# Autodesk Inventor assembly: FLUGGER POWER PNL ASSY
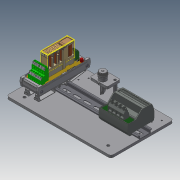
[picture p0: Inventor's stored thumbnail of the model, 180x180]
Saved by Autodesk Inventor 2020.3 (Build 243373000, 373)
## iProperties
RuleStatus: InUse
AfterDocSave0: file://Part Number Cleaner
Created: 2019-11-06
Vendor: HHMI: JRC - ID&F
Document SubType Name: Assembly
Designer: arnoldj
DESIGN DEPARTMENT: HHMI: JRC - ID&F
ALTERED ITEM PART NUMBER: N/A
ALTERED ITEM VENDOR: N/A
ALTERED ITEM DESCRIPTION: N/A
Author: arnoldj
Revision Number: 0
## Documents named in this file (9)
- C:\_WORKSPACE\DATA\PROJECTS\_PROJECTS BY LAB\CARD (LAB)\FLUGGER\FLUGGER POWER PNL ASSY.iam
- C:\_WORKSPACE\DATA\COMMON\Phoenix Contact\PHOENIX CONTACT 2315269 .ipt
- C:\_WORKSPACE\DATA\PROJECTS\_PROJECTS BY LAB\CARD (LAB)\FLUGGER\FLUGGER DIN RAIL MOUNT.ipt
- C:\_WORKSPACE\DATA\PROJECTS\_PROJECTS BY LAB\CARD (LAB)\FLUGGER\FLUGGER 8961K15 RAIL AI.ipt
- C:\_WORKSPACE\DATA\COMMON\Altech\Altech156.OA02.2433C.ipt
- C:\_WORKSPACE\DATA\PROJECTS\_PROJECTS BY LAB\CARD (LAB)\FLUGGER\FLUGGER FUSE MOUNT.ipt
- C:\_WORKSPACE\DATA\COMMON\McMaster\MCMASTER 7087K41 FUSEHOLDER .ipt
- C:\_WORKSPACE\DATA\COMMON\Littlefuse\Littlefuse 0218.315HXP.ipt
- C:\_WORKSPACE\DATA\COMMON\McMaster\MCMASTER 91115A146 STANDOFF 10-32x1_5L SS.ipt
## Components (9 placed, 8 different names)
1. FLUGGER DIN RAIL MOUNT:1 — Mate:1, Mate:2, Mate:3, Mate:4, Mate:7, Mate:10, Mate:11, Mate:12, Mate:16, Mate:18, Mate:19
2. PHOENIX CONTACT 2315269 :1 — Mate:5, Mate:6, Mate:7
3. FLUGGER 8961K15 RAIL AI:1 — Mate:1, Mate:2, Mate:3, Mate:4, Mate:5, Mate:6, Mate:8, Mate:9
4. Altech156.OA02.2433C:1 — Mate:8, Mate:9
5. FLUGGER FUSE MOUNT:1 — Mate:10, Mate:11, Mate:12, Mate:13, Mate:14, Mate:17
6. MCMASTER 7087K41 FUSEHOLDER :1 — Mate:13, Mate:14, Flush:1, Mate:15
7. Littlefuse 0218.315HXP:1 — Flush:1, Mate:15
8. MCMASTER 91115A146 STANDOFF 10-32x1_5L SS:1 — Mate:16, Mate:17
9. MCMASTER 91115A146 STANDOFF 10-32x1_5L SS:2 — Mate:18, Mate:19
## Relationships (20: Mate 19, Flush 1)
- Mate:1: FLUGGER DIN RAIL MOUNT:1 ↔ FLUGGER 8961K15 RAIL AI:1
- Mate:2: FLUGGER DIN RAIL MOUNT:1 ↔ FLUGGER 8961K15 RAIL AI:1
- Mate:3: FLUGGER DIN RAIL MOUNT:1 ↔ FLUGGER 8961K15 RAIL AI:1
- Mate:4: FLUGGER DIN RAIL MOUNT:1 ↔ FLUGGER 8961K15 RAIL AI:1
- Mate:5: PHOENIX CONTACT 2315269 :1 ↔ FLUGGER 8961K15 RAIL AI:1
- Mate:6: PHOENIX CONTACT 2315269 :1 ↔ FLUGGER 8961K15 RAIL AI:1
- Mate:7 (2.54 mm): FLUGGER DIN RAIL MOUNT:1 ↔ PHOENIX CONTACT 2315269 :1
- Mate:8: FLUGGER 8961K15 RAIL AI:1 ↔ Altech156.OA02.2433C:1
- Mate:9: FLUGGER 8961K15 RAIL AI:1 ↔ Altech156.OA02.2433C:1
- Mate:10 (38.1 mm): FLUGGER DIN RAIL MOUNT:1 ↔ FLUGGER FUSE MOUNT:1
- Mate:11: FLUGGER DIN RAIL MOUNT:1 ↔ FLUGGER FUSE MOUNT:1
- Mate:12: FLUGGER DIN RAIL MOUNT:1 ↔ FLUGGER FUSE MOUNT:1
- Mate:13: FLUGGER FUSE MOUNT:1 ↔ MCMASTER 7087K41 FUSEHOLDER :1
- Mate:14: FLUGGER FUSE MOUNT:1 ↔ MCMASTER 7087K41 FUSEHOLDER :1
- Flush:1: MCMASTER 7087K41 FUSEHOLDER :1 ↔ Littlefuse 0218.315HXP:1
- Mate:15: MCMASTER 7087K41 FUSEHOLDER :1 ↔ Littlefuse 0218.315HXP:1
- Mate:16: FLUGGER DIN RAIL MOUNT:1 ↔ MCMASTER 91115A146 STANDOFF 10-32x1_5L SS:1
- Mate:17: FLUGGER FUSE MOUNT:1 ↔ MCMASTER 91115A146 STANDOFF 10-32x1_5L SS:1
- Mate:18: FLUGGER DIN RAIL MOUNT:1 ↔ MCMASTER 91115A146 STANDOFF 10-32x1_5L SS:2
- Mate:19: FLUGGER DIN RAIL MOUNT:1 ↔ MCMASTER 91115A146 STANDOFF 10-32x1_5L SS:2
